# Autodesk Inventor assembly: SRassembly
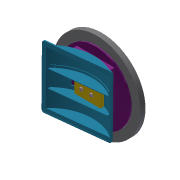
[picture p0: Inventor's stored thumbnail of the model, 180x180]
Saved by Autodesk Inventor 2022 Beta2 (Build 260130000, 130) ContinuousBuild 0
## iProperties
Created: 2010-03-04
Part Number: SRassembly
Document SubType Name: Assembly
Designer: jmacmillan
Author: jmacmillan
## Documents named in this file (7)
- C:\Autodesk Inventor 2021 Intro Practice Files\SRassembly_final.iam
- C:\Autodesk Inventor 2021 Intro Practice Files\SRbase.ipt
- C:\Autodesk Inventor 2021 Intro Practice Files\SRturntable.ipt
- C:\Autodesk Inventor 2021 Intro Practice Files\SRlocator.ipt
- C:\Autodesk Inventor 2021 Intro Practice Files\SRrocker.ipt
- C:\Autodesk Inventor 2021 Intro Practice Files\SRscrew.ipt
- C:\Autodesk Inventor 2021 Intro Practice Files\SRwasher.ipt
## Components (8 placed, 6 different names)
1. SRbase:1 — Insert:1, Angle:1, Insert:6
2. SRturntable:1 — Insert:1, Angle:1, Mate:1, Mate:2, Mate:3, Insert:2, Insert:3
3. SRlocator:1 — Insert:2, Insert:3, Insert:4, Insert:5
4. SRrocker:1 — Mate:1, Mate:2, Mate:3
5. SRscrew:1 — Insert:4
6. SRwasher:1 — Insert:6, Insert:7
7. SRscrew:2 — Insert:5
8. SRscrew:3 — Insert:7
## Relationships (11: Insert 7, Mate 3, Angle 1)
- Insert:1: SRbase:1 ↔ SRturntable:1
- Angle:1 (0 deg): SRbase:1 ↔ SRturntable:1
- Mate:1: SRturntable:1 ↔ SRrocker:1
- Mate:2: SRturntable:1 ↔ SRrocker:1
- Mate:3: SRturntable:1 ↔ SRrocker:1
- Insert:2: SRturntable:1 ↔ SRlocator:1
- Insert:3: SRturntable:1 ↔ SRlocator:1
- Insert:4: SRlocator:1 ↔ SRscrew:1
- Insert:5: SRlocator:1 ↔ SRscrew:2
- Insert:6: SRbase:1 ↔ SRwasher:1
- Insert:7: SRwasher:1 ↔ SRscrew:3
